# Autodesk Inventor assembly: Llantas y base
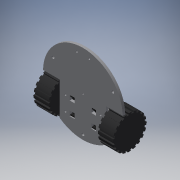
[picture p0: Inventor's stored thumbnail of the model, 180x180]
Saved by Autodesk Inventor 2017 (Build 210142000, 142)
## iProperties
Part Number: Llantas y base
Material: Genérico
Document SubType Name: Assembly
Designer: fam
Author: fam
## Documents named in this file (3)
- C:\Users\fam\Desktop\UVG\Ciclo 9\Megaproyecto\Megaproyecto\Diseños Inventor Fase 2\Llantas y base.iam
- C:\Users\fam\Desktop\UVG\Ciclo 9\Megaproyecto\Megaproyecto\Diseños Inventor Fase 2\Base.ipt
- C:\Users\fam\Desktop\UVG\Ciclo 9\Megaproyecto\Megaproyecto\Diseños Inventor Fase 2\Encoder-Motor-Llanta.iam
## Components (3 placed, 2 different names)
1. Base:1 — Coincidencia:1, Coincidencia:2, Coincidencia:3, Coincidencia:4, Coincidencia:5, Coincidencia:6
2. Encoder-Motor-Llanta:1 [sub-assembly] — Coincidencia:1, Coincidencia:2, Coincidencia:3
3. Encoder-Motor-Llanta:2 [sub-assembly] — Coincidencia:4, Coincidencia:5, Coincidencia:6
## Relationships (6: Mate 6)
- Coincidencia:1 [Mate]: Base:1 ↔ Encoder-Motor-Llanta:1
- Coincidencia:2 [Mate]: Base:1 ↔ Encoder-Motor-Llanta:1
- Coincidencia:3 [Mate]: Base:1 ↔ Encoder-Motor-Llanta:1
- Coincidencia:4 [Mate]: Base:1 ↔ Encoder-Motor-Llanta:2
- Coincidencia:5 [Mate]: Base:1 ↔ Encoder-Motor-Llanta:2
- Coincidencia:6 [Mate]: Base:1 ↔ Encoder-Motor-Llanta:2
